# Autodesk Inventor assembly: 14_outerlegg_assembly
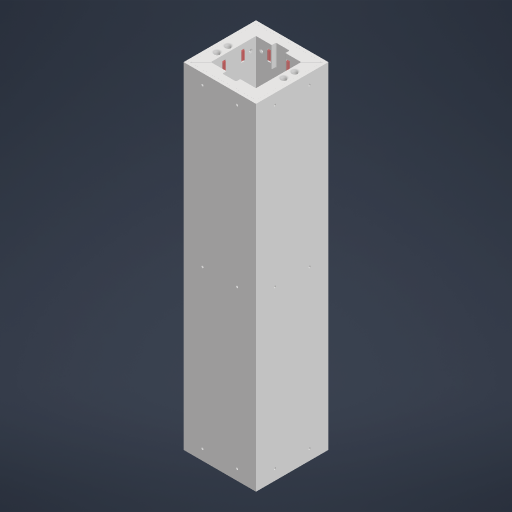
[picture p0: Inventor's stored thumbnail of the model, 512x512]
Saved by Autodesk Inventor 2024 (Build 280153000, 153)
## iProperties
Created: 2023-05-24
Part Number: 14_outerlegg_assembly
Document SubType Name: Assembly
Designer: aasmu
Author: aasmu
## Documents named in this file (5)
- C:\Users\aasmu\Documents\standing_desk\14_outerlegg_assembly.iam
- C:\Users\aasmu\Documents\standing_desk\outer_glide_carriage\11_outer_carriage_with_cable_roller.iam
- C:\Users\aasmu\Documents\standing_desk\outer_glide_carriage\12_outer_carriage_with_cable_pass_trough.iam
- C:\Users\aasmu\Documents\standing_desk\11_outerlegg_long_side.ipt
- C:\Users\aasmu\Documents\standing_desk\10_outerlegg_short_side.ipt
## Components (7 placed, 4 different names)
1. 11_outer_carriage_with_cable_roller:1 [sub-assembly] — Rigid:2
2. 12_outer_carriage_with_cable_pass_trough:1 [sub-assembly] — Rigid:1
3. 12_outer_carriage_with_cable_pass_trough:2 [sub-assembly] — Rigid:3, Rigid:4, Rigid:5, Rigid:6
4. 11_outerlegg_long_side:1 — Rigid:4
5. 11_outerlegg_long_side:2 — Rigid:5
6. 10_outerlegg_short_side:1 — Rigid:6
7. 10_outerlegg_short_side:2 — Rigid:1, Rigid:2, Rigid:3
## Relationships (6: WeldJoint 6)
- Rigid:1 [WeldJoint]: 12_outer_carriage_with_cable_pass_trough:1 ↔ 10_outerlegg_short_side:2
- Rigid:2 [WeldJoint]: 11_outer_carriage_with_cable_roller:1 ↔ 10_outerlegg_short_side:2
- Rigid:3 [WeldJoint]: 12_outer_carriage_with_cable_pass_trough:2 ↔ 10_outerlegg_short_side:2
- Rigid:4 [WeldJoint]: 12_outer_carriage_with_cable_pass_trough:2 ↔ 11_outerlegg_long_side:1
- Rigid:5 [WeldJoint]: 12_outer_carriage_with_cable_pass_trough:2 ↔ 11_outerlegg_long_side:2
- Rigid:6 [WeldJoint]: 12_outer_carriage_with_cable_pass_trough:2 ↔ 10_outerlegg_short_side:1
